# Autodesk Inventor assembly: złożenie przekładni prawa
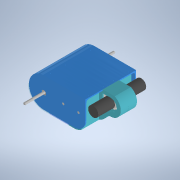
[picture p0: Inventor's stored thumbnail of the model, 180x180]
Saved by Autodesk Inventor 2021 (Build 250183000, 183)
## iProperties
Created: 2021-06-25
Part Number: złożenie przekładni prawa
Document SubType Name: Assembly
Designer: Łukasz
Author: Łukasz
## Documents named in this file (32)
- E:\GITHUB_Czołg\Szybki-Czolg-antyRadziecki\złożenie przekładni prawa.iam
- E:\GITHUB_Czołg\Szybki-Czolg-antyRadziecki\obudowa przekładni.ipt
- C:\Users\Łukasz\Documents\Inventor\Content Center Files\R2021\en-US\BS 292 (I)\BS 292 Part 1 - 608 - 8 x 22 x 7.ipt
- E:\GITHUB_Czołg\Szybki-Czolg-antyRadziecki\oś napędowa.ipt
- E:\GITHUB_Czołg\Szybki-Czolg-antyRadziecki\oś 8mm x 91mm.ipt
- E:\GITHUB_Czołg\Szybki-Czolg-antyRadziecki\koła zębate\Design Accelerator\inny set zebow\Design Accelerator\Spur Gear11.ipt
- E:\GITHUB_Czołg\Szybki-Czolg-antyRadziecki\koła zębate\Design Accelerator\podwojne koło zebate.iam
- E:\GITHUB_Czołg\Szybki-Czolg-antyRadziecki\koła zębate\Design Accelerator\podwojne koło zebate drugi skręt.iam
- E:\GITHUB_Czołg\Szybki-Czolg-antyRadziecki\koła zębate\Design Accelerator\inny set zebow\Design Accelerator\napędowy 40 zębow.ipt
- E:\GITHUB_Czołg\Szybki-Czolg-antyRadziecki\inne zęby\Design Accelerator\Spur Gear22.ipt
- E:\GITHUB_Czołg\Szybki-Czolg-antyRadziecki\silnik 3660.ipt
- E:\GITHUB_Czołg\Szybki-Czolg-antyRadziecki\koła zębate\Design Accelerator\inny set zebow\Design Accelerator\Spur Gear11 motor.ipt
- E:\GITHUB_Czołg\Szybki-Czolg-antyRadziecki\obudowa przekładni 2.ipt
- E:\GITHUB_Czołg\Szybki-Czolg-antyRadziecki\obudowa przekładni 3.ipt
- E:\GITHUB_Czołg\Szybki-Czolg-antyRadziecki\obudowa przekładni 4.ipt
- E:\GITHUB_Czołg\Szybki-Czolg-antyRadziecki\obudowa przekładni 5.ipt
- E:\GITHUB_Czołg\Szybki-Czolg-antyRadziecki\obudowa przekładni 6.ipt
- E:\GITHUB_Czołg\Szybki-Czolg-antyRadziecki\obudowa przekładni_MIR.ipt
- E:\GITHUB_Czołg\Szybki-Czolg-antyRadziecki\oś napędowa_MIR.ipt
- E:\GITHUB_Czołg\Szybki-Czolg-antyRadziecki\oś 8mm x 91mm_MIR.ipt
- E:\GITHUB_Czołg\Szybki-Czolg-antyRadziecki\koła zębate\Design Accelerator\inny set zebow\Design Accelerator\Spur Gear11_MIR.ipt
- E:\GITHUB_Czołg\Szybki-Czolg-antyRadziecki\koła zębate\Design Accelerator\podwojne koło zebate_MIR.iam
- E:\GITHUB_Czołg\Szybki-Czolg-antyRadziecki\koła zębate\Design Accelerator\podwojne koło zebate drugi skręt_MIR.iam
- E:\GITHUB_Czołg\Szybki-Czolg-antyRadziecki\koła zębate\Design Accelerator\inny set zebow\Design Accelerator\napędowy 40 zębow_MIR.ipt
- E:\GITHUB_Czołg\Szybki-Czolg-antyRadziecki\inne zęby\Design Accelerator\Spur Gear22_MIR.ipt
- E:\GITHUB_Czołg\Szybki-Czolg-antyRadziecki\silnik 3660_MIR.ipt
- E:\GITHUB_Czołg\Szybki-Czolg-antyRadziecki\koła zębate\Design Accelerator\inny set zebow\Design Accelerator\Spur Gear11 motor_MIR.ipt
- E:\GITHUB_Czołg\Szybki-Czolg-antyRadziecki\obudowa przekładni 2_MIR.ipt
- E:\GITHUB_Czołg\Szybki-Czolg-antyRadziecki\obudowa przekładni 3_MIR.ipt
- E:\GITHUB_Czołg\Szybki-Czolg-antyRadziecki\obudowa przekładni 4_MIR.ipt
- E:\GITHUB_Czołg\Szybki-Czolg-antyRadziecki\obudowa przekładni 5_MIR.ipt
- E:\GITHUB_Czołg\Szybki-Czolg-antyRadziecki\obudowa przekładni 6_MIR.ipt
## Components (60 placed, 29 different names)
1. obudowa przekładni:1 — Rotational:14, Rotational:15, Rigid:16, Rotational:16, Rotational:17, Rotational:18, Flush:2, Mate:1, Mate:2, Flush:3, Mate:3, Mate:4, Flush:6, Mate:6, Flush:7, Mate:8, Flush:8, Mate:10
2. BS 292: Part 1 (I) (Metric) 608 - 8 x 22 x 7:2 — Rotational:3, Rotational:5, Rotational:15
3. BS 292: Part 1 (I) (Metric) 608 - 8 x 22 x 7:1 — Rotational:14
4. oś napędowa:1 — Rotational:3, Rigid:15
5. oś 8mm x 91mm:1 — Rigid:16
6. Spur Gear1:1 — Rotational:4, Rotation:1, Rotational:7, Rotation:6, Rotational:17
7. podwojne koło zebate:1 [sub-assembly] — Rigid:4, Rigid:5, Rotation:1, Rotation:2
8. podwojne koło zebate:3 [sub-assembly] — Rigid:8, Rigid:9, Rotation:3, Rotation:4
9. BS 292: Part 1 (I) (Metric) 608 - 8 x 22 x 7:3 — Rotational:4
10. BS 292: Part 1 (I) (Metric) 608 - 8 x 22 x 7:4 — Rigid:4, Rotational:5
11. BS 292: Part 1 (I) (Metric) 608 - 8 x 22 x 7:5 — Rigid:5, Rotational:8
12. BS 292: Part 1 (I) (Metric) 608 - 8 x 22 x 7:6 — Rotational:7, Rotational:9
13. BS 292: Part 1 (I) (Metric) 608 - 8 x 22 x 7:7 — Rigid:12, Rotational:10
14. BS 292: Part 1 (I) (Metric) 608 - 8 x 22 x 7:8 — Rigid:8, Rotational:8
15. BS 292: Part 1 (I) (Metric) 608 - 8 x 22 x 7:9 — Rigid:9
16. BS 292: Part 1 (I) (Metric) 608 - 8 x 22 x 7:10 — Rigid:13, Rotational:10
17. BS 292: Part 1 (I) (Metric) 608 - 8 x 22 x 7:11 — Rigid:14
18. podwojne koło zebate drugi skręt:1 [sub-assembly] — Rigid:12, Rotational:9, Rotation:2, Rotation:3
19. podwojne koło zebate drugi skręt:2 [sub-assembly] — Rigid:13, Rigid:14, Rotation:4, Rotation:5
20. Spur Gear2:1 — Rigid:15, Rotation:5
21. oś 8mm x 91mm:2 — Rotational:16
22. Spur Gear2:2 — Rotational:11, Rotation:6, Flush:1, Tangent:1, Rotational:18, obrot silnika
23. BS 292: Part 1 (I) (Metric) 608 - 8 x 22 x 7:12 — Rotational:11
24. silnik 3660:1 — Flush:1, Tangent:1, Rotational:19
25. Spur Gear1:2 — Rotational:19, obrot silnika
26. obudowa przekładni 2:1 — Flush:2, Mate:1, Mate:2
27. obudowa przekładni 3:1 — Flush:3, Mate:3, Mate:4, Mate:7, Flush:9, Mate:9
28. obudowa przekładni 4:1 — Flush:6, Mate:6, Mate:7
29. obudowa przekładni 5:1 — Flush:7, Mate:8, Flush:8
30. obudowa przekładni 6:1 — Flush:9, Mate:9, Mate:10
31. obudowa przekładni_MIR:1 — Mate:11, Mate:12, Flush:11, Mate:13, Mate:14, Flush:12, Flush:13, Mate:16, Flush:14, Mate:17, Flush:15, Mate:18, Rotational:20, Rotational:21, Rigid:17, Rotational:29
32. BS 292: Part 1 (I) (Metric) 608 - 8 x 22 x 7:13 — Rotational:20, Rotational:22, Rotational:24
33. BS 292: Part 1 (I) (Metric) 608 - 8 x 22 x 7:14 — Rotational:21
34. oś napędowa_MIR:1 — Rotational:22, Rigid:25
35. oś 8mm x 91mm_MIR:1 — Rigid:17
36. Spur Gear11_MIR:1 — Rotation:8, Rotation:13, Rotational:23, Rotational:25
37. podwojne koło zebate_MIR:1 [sub-assembly] — Rotation:8, Rotation:10, Rigid:18, Rigid:19
38. podwojne koło zebate_MIR:2 [sub-assembly] — Rotation:9, Rotation:11, Rigid:20, Rigid:21
39. BS 292: Part 1 (I) (Metric) 608 - 8 x 22 x 7:15 — Rotational:23
40. BS 292: Part 1 (I) (Metric) 608 - 8 x 22 x 7:16 — Rotational:24, Rigid:18
41. BS 292: Part 1 (I) (Metric) 608 - 8 x 22 x 7:17 — Rigid:19, Rotational:26
42. BS 292: Part 1 (I) (Metric) 608 - 8 x 22 x 7:18 — Rotational:25, Rotational:28
43. BS 292: Part 1 (I) (Metric) 608 - 8 x 22 x 7:19 — Rotational:27, Rigid:22
44. BS 292: Part 1 (I) (Metric) 608 - 8 x 22 x 7:20 — Rotational:26, Rigid:20
45. BS 292: Part 1 (I) (Metric) 608 - 8 x 22 x 7:21 — Rigid:21
46. BS 292: Part 1 (I) (Metric) 608 - 8 x 22 x 7:22 — Rotational:27, Rigid:24
47. BS 292: Part 1 (I) (Metric) 608 - 8 x 22 x 7:23 — Rigid:23
48. podwojne koło zebate drugi skręt_MIR:1 [sub-assembly] — Rotation:9, Rotation:10, Rotational:28, Rigid:22
49. podwojne koło zebate drugi skręt_MIR:2 [sub-assembly] — Rotation:11, Rotation:12, Rigid:23, Rigid:24
50. napędowy 40 zębow_MIR:1 — Rotation:12, Rigid:25
51. oś 8mm x 91mm_MIR:2 — Rotational:29
52. Spur Gear22_MIR:1 — Rotation:13, Tangent:2, Flush:10, Rotation:14, Rotational:30
53. BS 292: Part 1 (I) (Metric) 608 - 8 x 22 x 7:24 — Rotational:30
54. silnik 3660_MIR:1 — Tangent:2, Flush:10, Rotational:31
55. Spur Gear11 motor_MIR:1 — Rotation:14, Rotational:31
56. obudowa przekładni 2_MIR:1 — Mate:11, Mate:12, Flush:11
57. obudowa przekładni 3_MIR:1 — Mate:13, Mate:14, Flush:12, Mate:15, Mate:19, Flush:16
58. obudowa przekładni 4_MIR:1 — Mate:15, Flush:13, Mate:16
59. obudowa przekładni 5_MIR:1 — Flush:14, Mate:17, Flush:15
60. obudowa przekładni 6_MIR:1 — Mate:18, Mate:19, Flush:16
## Relationships (92: RevoluteJoint 26, WeldJoint 18, Mate 18, RelateRotation 14, Flush 14, Tangent 2)
- Rotational:3 [RevoluteJoint]: BS 292: Part 1 (I) (Metric) 608 - 8 x 22 x 7:2 ↔ oś napędowa:1
- Rotational:4 [RevoluteJoint] (-3.5 mm): Spur Gear1:1 ↔ BS 292: Part 1 (I) (Metric) 608 - 8 x 22 x 7:3
- Rigid:4 [WeldJoint]: podwojne koło zebate:1 ↔ BS 292: Part 1 (I) (Metric) 608 - 8 x 22 x 7:4
- Rigid:5 [WeldJoint]: podwojne koło zebate:1 ↔ BS 292: Part 1 (I) (Metric) 608 - 8 x 22 x 7:5
- Rigid:8 [WeldJoint]: podwojne koło zebate:3 ↔ BS 292: Part 1 (I) (Metric) 608 - 8 x 22 x 7:8
- Rigid:9 [WeldJoint]: podwojne koło zebate:3 ↔ BS 292: Part 1 (I) (Metric) 608 - 8 x 22 x 7:9
- Rotational:5 [RevoluteJoint] (2 mm): BS 292: Part 1 (I) (Metric) 608 - 8 x 22 x 7:2 ↔ BS 292: Part 1 (I) (Metric) 608 - 8 x 22 x 7:4
- Rotation:1 [RelateRotation] (2 ul): Spur Gear1:1 ↔ podwojne koło zebate:1
- Rotational:7 [RevoluteJoint] (-2 mm): Spur Gear1:1 ↔ BS 292: Part 1 (I) (Metric) 608 - 8 x 22 x 7:6
- Rotational:8 [RevoluteJoint] (2 mm): BS 292: Part 1 (I) (Metric) 608 - 8 x 22 x 7:5 ↔ BS 292: Part 1 (I) (Metric) 608 - 8 x 22 x 7:8
- Rigid:12 [WeldJoint]: BS 292: Part 1 (I) (Metric) 608 - 8 x 22 x 7:7 ↔ podwojne koło zebate drugi skręt:1
- Rotational:9 [RevoluteJoint]: BS 292: Part 1 (I) (Metric) 608 - 8 x 22 x 7:6 ↔ podwojne koło zebate drugi skręt:1
- Rotation:2 [RelateRotation] (2 ul): podwojne koło zebate:1 ↔ podwojne koło zebate drugi skręt:1
- Rotation:3 [RelateRotation] (2 ul): podwojne koło zebate:3 ↔ podwojne koło zebate drugi skręt:1
- Rigid:13 [WeldJoint]: BS 292: Part 1 (I) (Metric) 608 - 8 x 22 x 7:10 ↔ podwojne koło zebate drugi skręt:2
- Rigid:14 [WeldJoint]: BS 292: Part 1 (I) (Metric) 608 - 8 x 22 x 7:11 ↔ podwojne koło zebate drugi skręt:2
- Rotational:10 [RevoluteJoint] (2 mm): BS 292: Part 1 (I) (Metric) 608 - 8 x 22 x 7:7 ↔ BS 292: Part 1 (I) (Metric) 608 - 8 x 22 x 7:10
- Rotation:4 [RelateRotation] (2 ul): podwojne koło zebate:3 ↔ podwojne koło zebate drugi skręt:2
- Rigid:15 [WeldJoint] (-23 mm): oś napędowa:1 ↔ Spur Gear2:1
- Rotation:5 [RelateRotation] (2 ul): podwojne koło zebate drugi skręt:2 ↔ Spur Gear2:1
- Rotational:11 [RevoluteJoint] (-1 mm): Spur Gear2:2 ↔ BS 292: Part 1 (I) (Metric) 608 - 8 x 22 x 7:12
- Rotation:6 [RelateRotation] (1.35 ul): Spur Gear1:1 ↔ Spur Gear2:2
- Flush:1 (16 mm): Spur Gear2:2 ↔ silnik 3660:1
- Tangent:1 (25 mm): Spur Gear2:2 ↔ silnik 3660:1
- Rotational:14 [RevoluteJoint]: obudowa przekładni:1 ↔ BS 292: Part 1 (I) (Metric) 608 - 8 x 22 x 7:1
- Rotational:15 [RevoluteJoint]: obudowa przekładni:1 ↔ BS 292: Part 1 (I) (Metric) 608 - 8 x 22 x 7:2
- Rigid:16 [WeldJoint]: obudowa przekładni:1 ↔ oś 8mm x 91mm:1
- Rotational:16 [RevoluteJoint]: obudowa przekładni:1 ↔ oś 8mm x 91mm:2
- Rotational:17 [RevoluteJoint] (2 mm): obudowa przekładni:1 ↔ Spur Gear1:1
- Rotational:18 [RevoluteJoint] (2 mm): obudowa przekładni:1 ↔ Spur Gear2:2
- Rotational:19 [RevoluteJoint]: silnik 3660:1 ↔ Spur Gear1:2
- obrot silnika [RelateRotation] (1.35 ul): Spur Gear2:2 ↔ Spur Gear1:2
- Flush:2: obudowa przekładni:1 ↔ obudowa przekładni 2:1
- Mate:1: obudowa przekładni:1 ↔ obudowa przekładni 2:1
- Mate:2: obudowa przekładni:1 ↔ obudowa przekładni 2:1
- Flush:3: obudowa przekładni:1 ↔ obudowa przekładni 3:1
- Mate:3: obudowa przekładni:1 ↔ obudowa przekładni 3:1
- Mate:4: obudowa przekładni:1 ↔ obudowa przekładni 3:1
- Flush:6: obudowa przekładni:1 ↔ obudowa przekładni 4:1
- Mate:6: obudowa przekładni:1 ↔ obudowa przekładni 4:1
- Mate:7: obudowa przekładni 3:1 ↔ obudowa przekładni 4:1
- Flush:7: obudowa przekładni:1 ↔ obudowa przekładni 5:1
- Mate:8: obudowa przekładni:1 ↔ obudowa przekładni 5:1
- Flush:8: obudowa przekładni:1 ↔ obudowa przekładni 5:1
- Flush:9: obudowa przekładni 3:1 ↔ obudowa przekładni 6:1
- Mate:9: obudowa przekładni 3:1 ↔ obudowa przekładni 6:1
- Mate:10: obudowa przekładni:1 ↔ obudowa przekładni 6:1
- Rotation:8 [RelateRotation] (2 ul): Spur Gear11_MIR:1 ↔ podwojne koło zebate_MIR:1
- Rotation:9 [RelateRotation] (2 ul): podwojne koło zebate_MIR:2 ↔ podwojne koło zebate drugi skręt_MIR:1
- Rotation:10 [RelateRotation] (2 ul): podwojne koło zebate_MIR:1 ↔ podwojne koło zebate drugi skręt_MIR:1
- Rotation:11 [RelateRotation] (2 ul): podwojne koło zebate_MIR:2 ↔ podwojne koło zebate drugi skręt_MIR:2
- Rotation:12 [RelateRotation] (2 ul): podwojne koło zebate drugi skręt_MIR:2 ↔ napędowy 40 zębow_MIR:1
- Rotation:13 [RelateRotation] (1.35 ul): Spur Gear11_MIR:1 ↔ Spur Gear22_MIR:1
- Tangent:2 (25 mm): Spur Gear22_MIR:1 ↔ silnik 3660_MIR:1
- Flush:10 (16 mm): Spur Gear22_MIR:1 ↔ silnik 3660_MIR:1
- Rotation:14 [RelateRotation] (1.35 ul): Spur Gear22_MIR:1 ↔ Spur Gear11 motor_MIR:1
- Mate:11: obudowa przekładni_MIR:1 ↔ obudowa przekładni 2_MIR:1
- Mate:12: obudowa przekładni_MIR:1 ↔ obudowa przekładni 2_MIR:1
- Flush:11: obudowa przekładni_MIR:1 ↔ obudowa przekładni 2_MIR:1
- Mate:13: obudowa przekładni_MIR:1 ↔ obudowa przekładni 3_MIR:1
- Mate:14: obudowa przekładni_MIR:1 ↔ obudowa przekładni 3_MIR:1
- Flush:12: obudowa przekładni_MIR:1 ↔ obudowa przekładni 3_MIR:1
- Mate:15: obudowa przekładni 3_MIR:1 ↔ obudowa przekładni 4_MIR:1
- Flush:13: obudowa przekładni_MIR:1 ↔ obudowa przekładni 4_MIR:1
- Mate:16: obudowa przekładni_MIR:1 ↔ obudowa przekładni 4_MIR:1
- Flush:14: obudowa przekładni_MIR:1 ↔ obudowa przekładni 5_MIR:1
- Mate:17: obudowa przekładni_MIR:1 ↔ obudowa przekładni 5_MIR:1
- Flush:15: obudowa przekładni_MIR:1 ↔ obudowa przekładni 5_MIR:1
- Mate:18: obudowa przekładni_MIR:1 ↔ obudowa przekładni 6_MIR:1
- Mate:19: obudowa przekładni 3_MIR:1 ↔ obudowa przekładni 6_MIR:1
- Flush:16: obudowa przekładni 3_MIR:1 ↔ obudowa przekładni 6_MIR:1
- Rotational:20 [RevoluteJoint]: obudowa przekładni_MIR:1 ↔ BS 292: Part 1 (I) (Metric) 608 - 8 x 22 x 7:13
- Rotational:21 [RevoluteJoint]: obudowa przekładni_MIR:1 ↔ BS 292: Part 1 (I) (Metric) 608 - 8 x 22 x 7:14
- Rotational:22 [RevoluteJoint]: BS 292: Part 1 (I) (Metric) 608 - 8 x 22 x 7:13 ↔ oś napędowa_MIR:1
- Rigid:17 [WeldJoint]: obudowa przekładni_MIR:1 ↔ oś 8mm x 91mm_MIR:1
- Rotational:23 [RevoluteJoint] (3.5 mm): Spur Gear11_MIR:1 ↔ BS 292: Part 1 (I) (Metric) 608 - 8 x 22 x 7:15
- Rotational:24 [RevoluteJoint] (2 mm): BS 292: Part 1 (I) (Metric) 608 - 8 x 22 x 7:13 ↔ BS 292: Part 1 (I) (Metric) 608 - 8 x 22 x 7:16
- Rigid:18 [WeldJoint]: podwojne koło zebate_MIR:1 ↔ BS 292: Part 1 (I) (Metric) 608 - 8 x 22 x 7:16
- Rigid:19 [WeldJoint]: podwojne koło zebate_MIR:1 ↔ BS 292: Part 1 (I) (Metric) 608 - 8 x 22 x 7:17
- Rotational:25 [RevoluteJoint] (2 mm): Spur Gear11_MIR:1 ↔ BS 292: Part 1 (I) (Metric) 608 - 8 x 22 x 7:18
- Rotational:26 [RevoluteJoint] (2 mm): BS 292: Part 1 (I) (Metric) 608 - 8 x 22 x 7:17 ↔ BS 292: Part 1 (I) (Metric) 608 - 8 x 22 x 7:20
- Rigid:20 [WeldJoint]: podwojne koło zebate_MIR:2 ↔ BS 292: Part 1 (I) (Metric) 608 - 8 x 22 x 7:20
- Rigid:21 [WeldJoint]: podwojne koło zebate_MIR:2 ↔ BS 292: Part 1 (I) (Metric) 608 - 8 x 22 x 7:21
- Rotational:27 [RevoluteJoint] (2 mm): BS 292: Part 1 (I) (Metric) 608 - 8 x 22 x 7:19 ↔ BS 292: Part 1 (I) (Metric) 608 - 8 x 22 x 7:22
- Rotational:28 [RevoluteJoint]: BS 292: Part 1 (I) (Metric) 608 - 8 x 22 x 7:18 ↔ podwojne koło zebate drugi skręt_MIR:1
- Rigid:22 [WeldJoint]: BS 292: Part 1 (I) (Metric) 608 - 8 x 22 x 7:19 ↔ podwojne koło zebate drugi skręt_MIR:1
- Rigid:23 [WeldJoint]: BS 292: Part 1 (I) (Metric) 608 - 8 x 22 x 7:23 ↔ podwojne koło zebate drugi skręt_MIR:2
- Rigid:24 [WeldJoint]: BS 292: Part 1 (I) (Metric) 608 - 8 x 22 x 7:22 ↔ podwojne koło zebate drugi skręt_MIR:2
- Rigid:25 [WeldJoint] (23 mm): oś napędowa_MIR:1 ↔ napędowy 40 zębow_MIR:1
- Rotational:29 [RevoluteJoint]: obudowa przekładni_MIR:1 ↔ oś 8mm x 91mm_MIR:2
- Rotational:30 [RevoluteJoint] (1 mm): Spur Gear22_MIR:1 ↔ BS 292: Part 1 (I) (Metric) 608 - 8 x 22 x 7:24
- Rotational:31 [RevoluteJoint]: silnik 3660_MIR:1 ↔ Spur Gear11 motor_MIR:1
